# Autodesk Inventor assembly: 1 cell.Tube and Pipe Runs10
(part 2 of 2)
Elbow45Key: v3#421a8b99-1721-409a-bc3b-c00889561754#1
_ComponentInfo: <CS><C N="Pipe" R="2.000000" IR="1.950000" PL="PL" PN="ISO 4065 Pipe 40 x 0.5 S40"><CO N="1"><FE V="0"/><FD V="0"/><ET V="Jointed"/><NS V="M40"/><MA  V="6.000000"/><MI V="1.200000"/><WP X="25.000000" Y="0.000000" Z="0.000000"/><WA X="1.000000" Y="0.000000" Z="0.000000"/></CO><CO N="2"><FE  V="0"/><FD V="1"/><ET V="Jointed"/><NS V="M40"/><MA V="6.000000"/><MI V="1.200000"/><WP X="0.000000" Y="0.000000" Z="0.000000"/><WA X="1.000000"  Y="0.000000" Z="0.000000"/></CO></C><C N="Coupling" CW="7.660000"><CO N="1"><FE V="1"/><FD V="1"/><ET V="Jointed"/><NS V="M40"/><MA V="3.830000"/><MI  V="0.766000"/><WP X="-0.000000" Y="0.000000" Z="0.000000"/><WA X="-1.000000" Y="0.000000" Z="0.000000"/></CO><CO N="2"><FE V="1"/><FD V="0"/><ET  V="Jointed"/><NS V="M40"/><MA V="3.830000"/><MI V="0.766000"/><WP X="-7.660000" Y="0.000000" Z="0.000000"/><WA X="-1.000000" Y="0.000000"  Z="0.000000"/></CO></C><C N="Elbow90" ER="3.850394" S1="7.450394" S2="7.450394" D1="3.600000" D2="3.600000"><CO N="1"><FE V="1"/><FD V="1"/><ET  V="Jointed"/><NS V="M40"/><MA V="3.600000"/><MI V="0.720000"/><WP X="7.450394" Y="0.000000" Z="7.450394"/><WA X="-1.000000" Y="0.000000"  Z="0.000000"/></CO><CO N="2"><FE V="1"/><FD V="0"/><ET V="Jointed"/><NS V="M40"/><MA V="3.600000"/><MI V="0.720000"/><WP X="-0.000000" Y="0.000000"  Z="0.000000"/><WA X="0.000000" Y="0.000000" Z="-1.000000"/></CO></C><C N="Elbow45" ER="5.674352" S1="5.950394" S2="5.950394" D1="3.600000"  D2="3.600000"><CO N="1"><FE V="1"/><FD V="1"/><ET V="Jointed"/><NS V="M40"/><MA V="3.600000"/><MI V="0.720000"/><WP X="4.207564" Y="0.000000"  Z="10.157957"/><WA X="-0.707107" Y="0.000000" Z="-0.707107"/></CO><CO N="2"><FE V="1"/><FD V="0"/><ET V="Jointed"/><NS V="M40"/><MA V="3.600000"/><MI  V="0.720000"/><WP X="-0.000000" Y="0.000000" Z="0.000000"/><WA X="0.000000" Y="0.000000" Z="-1.000000"/></CO></C></CS>
Angle: UnInitValue
IsSelfDraining: UnInitValue
Author: a.komeijani
Name: Hydraulic Hose - No Fittings
SuppressStartFitting: True
SuppressEndFitting: True
## Documents named in this file (10)
- E:\my-aquaponic\Inventor\1 cell\AIP\Tube and Pipe\1 cell.Tube and Pipe Runs10.iam
- E:\my-aquaponic\Inventor\1 cell\AIP\Tube and Pipe\Run18\1 cell.Run18.iam
- E:\my-aquaponic\Inventor\1 cell\AIP\Tube and Pipe\Run19\1 cell.Run19.iam
- E:\my-aquaponic\Inventor\1 cell\AIP\Tube and Pipe\Run21\1 cell.Run21.iam
- C:\Users\a.komeijani\Documents\Inventor\Content Center Files\R2020\en-US\ASTM D 2466(2)\ASTM D 2466 Reducer Bushing Socket-Type 1 - Schedule 40 4 x 2.ipt
- E:\my-aquaponic\Inventor\1 cell\AIP\Tube and Pipe\Run22\1 cell.Run22.iam
- C:\Users\a.komeijani\Documents\Inventor\Content Center Files\R2020\en-US\ISO 3633 45 (08)\ISO 3633 90 Deg Bend with Only Sockets for Cemented Type Joints DN63.ipt
- E:\my-aquaponic\Inventor\1 cell\AIP\Tube and Pipe\Run23\1 cell.Run23.iam
- E:\my-aquaponic\Inventor\1 cell\AIP\Tube and Pipe\Run24\1 cell.Run24.iam
- E:\my-aquaponic\Inventor\1 cell\AIP\Tube and Pipe\Run25\1 cell.Run25.iam
## Components (11 placed, 9 different names)
1. Run18 [sub-assembly]
2. Run19 [sub-assembly] — Insert:3
3. Run21 [sub-assembly]
4. ASTM D 2466 Reducer Bushing Socket-Type 1 - Schedule 40 4 x 2:1 — Insert:1
5. Run22 [sub-assembly] — Insert:1, Insert:2
6. ISO 3633 90 Deg Bend with Only Sockets for Cemented Type Joints DN63:1
7. ISO 3633 90 Deg Bend with Only Sockets for Cemented Type Joints DN63:2 — Insert:2
8. ISO 3633 90 Deg Bend with Only Sockets for Cemented Type Joints DN63:3 — Insert:3
9. Run23 [sub-assembly]
10. Run24 [sub-assembly]
11. Run25 [sub-assembly]
## Relationships (3: Insert 3)
- Insert:1 (-80 mm): ASTM D 2466 Reducer Bushing Socket-Type 1 - Schedule 40 4 x 2:1 ↔ Run22
- Insert:2: Run22 ↔ ISO 3633 90 Deg Bend with Only Sockets for Cemented Type Joints DN63:2
- Insert:3: Run19 ↔ ISO 3633 90 Deg Bend with Only Sockets for Cemented Type Joints DN63:3
